# Autodesk Inventor assembly: assembly
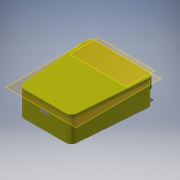
[picture p0: Inventor's stored thumbnail of the model, 180x180]
Saved by Autodesk Inventor 2019 (Build 230136000, 136)
## iProperties
Created: 2020-06-11
Part Number: assembly
Document SubType Name: Assembly
Designer: assman
Author: assman
## Documents named in this file (4)
- D:\Inventor\Projects\PS2ToJoystick\assembly.iam
- D:\Inventor\Projects\3party\Boards\ArduinoMicro\microplaceholder.ipt
- D:\Inventor\Projects\PS2ToJoystick\ps2conn.ipt
- D:\Inventor\Projects\PS2ToJoystick\box.ipt
## Components (3 placed, 3 different names)
1. microplaceholder:1
2. ps2conn:1 — Flush:1, Flush:2
3. box:1 — Flush:3
## Relationships (3: Flush 3)
- Flush:1 (5 mm): ps2conn:1
- Flush:2 (5 mm): ps2conn:1
- Flush:3: box:1
